# Autodesk Inventor assembly: Optical Device Assembly
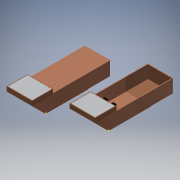
[picture p0: Inventor's stored thumbnail of the model, 180x180]
Saved by Autodesk Inventor 2017 (Build 210142000, 142)
## iProperties
Created: 2019-04-10
Part Number: Optical Device Assembly
Document SubType Name: Assembly
Designer: Sharat
Author: Sharat
## Documents named in this file (7)
- C:\Users\Sharat\Desktop\OpticalDeviceCAD\Optical Device Assembly.iam
- C:\Users\Sharat\Desktop\OpticalDeviceLensHolder.ipt
- C:\Users\Sharat\Desktop\OpticalDeviceLookThroughPart.ipt
- C:\Users\Sharat\Downloads\OpticalDeviceMirrorPart.ipt
- C:\Users\Sharat\Downloads\OpticalDeviceLensPart (1).ipt
- C:\Users\Sharat\Downloads\OpticalDeviceObjectPart.ipt
- C:\Users\Sharat\Desktop\OpticalDeviceRoof.ipt
## Components (11 placed, 6 different names)
1. OpticalDeviceLensHolder:1 — Mate:7, Mate:8
2. OpticalDeviceLookThroughPart:1 — Mate:5, Mate:6
3. OpticalDeviceLensPart (1):1 — Mate:1, Mate:2, Mate:3, Mate:4
4. OpticalDeviceMirrorPart:1 — Mate:3, Mate:4, Mate:5, Mate:6, Mate:7, Mate:8
5. OpticalDeviceObjectPart:1 — Mate:1, Mate:2
6. OpticalDeviceLensHolder:2
7. OpticalDeviceLookThroughPart:2
8. OpticalDeviceLensPart (1):2 — Mate:17, Mate:18
9. OpticalDeviceMirrorPart:2
10. OpticalDeviceObjectPart:2
11. OpticalDeviceRoof:1 — Mate:17, Mate:18
## Relationships (18: Mate 18)
- Mate:1: OpticalDeviceLensPart (1):1 ↔ OpticalDeviceObjectPart:1
- Mate:2: OpticalDeviceLensPart (1):1 ↔ OpticalDeviceObjectPart:1
- Mate:3: OpticalDeviceLensPart (1):1 ↔ OpticalDeviceMirrorPart:1
- Mate:4: OpticalDeviceLensPart (1):1 ↔ OpticalDeviceMirrorPart:1
- Mate:5: OpticalDeviceLookThroughPart:1 ↔ OpticalDeviceMirrorPart:1
- Mate:6: OpticalDeviceLookThroughPart:1 ↔ OpticalDeviceMirrorPart:1
- Mate:7: OpticalDeviceLensHolder:1 ↔ OpticalDeviceMirrorPart:1
- Mate:8: OpticalDeviceLensHolder:1 ↔ OpticalDeviceMirrorPart:1
- [Mate]: OpticalDeviceLensPart (1):2 ↔ OpticalDeviceObjectPart:2
- [Mate]: OpticalDeviceLensPart (1):2 ↔ OpticalDeviceObjectPart:2
- [Mate]: OpticalDeviceLensPart (1):2 ↔ OpticalDeviceMirrorPart:2
- [Mate]: OpticalDeviceLensPart (1):2 ↔ OpticalDeviceMirrorPart:2
- [Mate]: OpticalDeviceLookThroughPart:2 ↔ OpticalDeviceMirrorPart:2
- [Mate]: OpticalDeviceLookThroughPart:2 ↔ OpticalDeviceMirrorPart:2
- [Mate]: OpticalDeviceLensHolder:2 ↔ OpticalDeviceMirrorPart:2
- [Mate]: OpticalDeviceLensHolder:2 ↔ OpticalDeviceMirrorPart:2
- Mate:17: OpticalDeviceLensPart (1):2 ↔ OpticalDeviceRoof:1
- Mate:18: OpticalDeviceLensPart (1):2 ↔ OpticalDeviceRoof:1
## Named parameters: d12_d11 = 0 mm, d13_d4 = 0 mm, d14_d5 = 0 mm, d15_d6 = 0 mm, d16_d7 = 0 mm, d17_d8 = 0 mm, d18_d9 = 0 mm, d19_d10 = 0 mm
